# Autodesk Inventor assembly: 적재함_고정대_ASSEMBLY
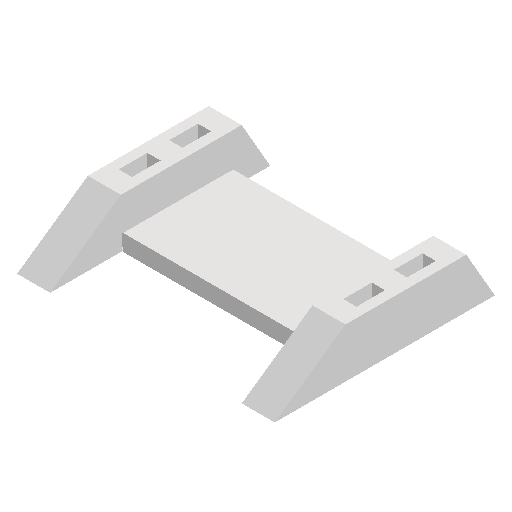
[picture p0: Inventor's stored thumbnail of the model, 512x512]
Saved by Autodesk Inventor 2027 (Build 310192000, 192)
## iProperties
Created: 2026-09-21
Part Number: 적재함_고정대_ASSEMBLY
Document SubType Name: Assembly
Designer: User
Author: User
## Documents named in this file (4)
- C:\Users\User\Desktop\4_권도영\졸업작품\INVENTOR\분류대_적재함\적재함_고정대_ASSEMBLY.iam
- C:\Users\User\Desktop\4_권도영\졸업작품\INVENTOR\분류대_적재함\적재함_부품_1.ipt
- C:\Users\User\Desktop\4_권도영\졸업작품\INVENTOR\분류대_적재함\적재함_부품_2.ipt
- C:\Users\User\Desktop\4_권도영\졸업작품\INVENTOR\분류대_적재함\브릿지.ipt
## Components (3 placed, 3 different names)
1. 적재함_부품_1:1 — 메이트:2, 플러쉬:2
2. 적재함_부품_2:1 — 메이트:1, 플러쉬:1
3. 브릿지:1 — 메이트:1, 플러쉬:1, 메이트:2, 플러쉬:2
## Relationships (4: Mate 2, Flush 2)
- 메이트:1 [Mate]: 적재함_부품_2:1 ↔ 브릿지:1
- 플러쉬:1 [Flush]: 적재함_부품_2:1 ↔ 브릿지:1
- 메이트:2 [Mate]: 적재함_부품_1:1 ↔ 브릿지:1
- 플러쉬:2 [Flush]: 적재함_부품_1:1 ↔ 브릿지:1
